# Autodesk Inventor assembly: Unit_SR-T
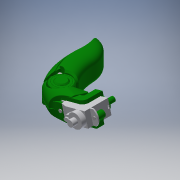
[picture p0: Inventor's stored thumbnail of the model, 180x180]
Saved by Autodesk Inventor 2018.2 (Build 222227000, 227)
## iProperties
Created: 2018-02-15
Part Number: Unit_SR-T
Material: 一般
Document SubType Name: Assembly
Designer: sktom
Author: sktom
Title: Unit_SR-T
## Documents named in this file (9)
- D:\CloudStrage\OneDrive\CADMech\HbSizeSMech\UnitHand\Unit_SR-H\Unit_SR-T\Unit_SR-T.iam
- D:\CloudStrage\OneDrive\CADMech\HbSizeSMech\UnitHand\Unit_SR-H\Unit_SR-T\SR-T-03.ipt
- D:\CloudStrage\OneDrive\CADMech\HbSizeSMech\UnitHand\Unit_SR-H\Unit_SR-T\SR-T-04.ipt
- D:\CloudStrage\OneDrive\CADMech\HbSizeSMech\UnitHand\Unit_SR-H\Unit_SR-T\SR-T-02.ipt
- D:\CloudStrage\OneDrive\CADMech\HbSizeSMech\UnitHand\Unit_SR-H\Unit_SR-T\SR-T-05.ipt
- D:\CloudStrage\OneDrive\CADMech\HbSizeSMech\UnitHand\Unit_SR-H\Unit_SR-T\SR-T-01.ipt
- D:\CloudStrage\OneDrive\CADMech\HbSizeSMech\UnitHand\Unit_SR-H\Unit_SR-T\Parts_Servo_HK282A.ipt
- D:\CloudStrage\OneDrive\CADMech\HbSizeSMech\UnitHand\Unit_SR-H\Unit_SR-T\SR-T-06.ipt
- D:\CloudStrage\OneDrive\CADMech\HbSizeSMech\UnitHand\Unit_SR-H\Unit_SR-T\Parts_Screw_M1.4_L6.ipt
## Components (13 placed, 8 different names)
1. SR-T-01 — 挿入:5, 挿入:9
2. SR-T-02 — 挿入:4, 挿入:5
3. SR-T-03 — 挿入:1, 挿入:2, 挿入:3, 挿入:4, 挿入:6, 挿入:7, 挿入:14
4. SR-T-04 — 挿入:3
5. SR-T-05 — 挿入:1, 挿入:2, 挿入:10, 挿入:11
6. SR-T-06 — 挿入:8, 挿入:12
7. Parts_Servo_HK282A:1 — 挿入:6, 挿入:7, 挿入:8, 挿入:13
8. Parts_Screw_M1.4_L6:1 — 挿入:9
9. Parts_Screw_M1.4_L6:2 — 挿入:10
10. Parts_Screw_M1.4_L6:3 — 挿入:11
11. Parts_Screw_M1.4_L6:4 — 挿入:12
12. Parts_Screw_M1.4_L6:5 — 挿入:13
13. Parts_Screw_M1.4_L6:6 — 挿入:14
## Relationships (14: Insert 14)
- 挿入:1 [Insert]: SR-T-03 ↔ SR-T-05
- 挿入:2 [Insert]: SR-T-03 ↔ SR-T-05
- 挿入:3 [Insert] (1 mm): SR-T-03 ↔ SR-T-04
- 挿入:4 [Insert] (0.1 mm): SR-T-02 ↔ SR-T-03
- 挿入:5 [Insert]: SR-T-01 ↔ SR-T-02
- 挿入:6 [Insert]: SR-T-03 ↔ Parts_Servo_HK282A:1
- 挿入:7 [Insert]: SR-T-03 ↔ Parts_Servo_HK282A:1
- 挿入:8 [Insert]: SR-T-06 ↔ Parts_Servo_HK282A:1
- 挿入:9 [Insert]: SR-T-01 ↔ Parts_Screw_M1.4_L6:1
- 挿入:10 [Insert]: SR-T-05 ↔ Parts_Screw_M1.4_L6:2
- 挿入:11 [Insert]: SR-T-05 ↔ Parts_Screw_M1.4_L6:3
- 挿入:12 [Insert]: SR-T-06 ↔ Parts_Screw_M1.4_L6:4
- 挿入:13 [Insert]: Parts_Servo_HK282A:1 ↔ Parts_Screw_M1.4_L6:5
- 挿入:14 [Insert]: SR-T-03 ↔ Parts_Screw_M1.4_L6:6
